# Autodesk Inventor assembly: Nozzle-Brush-Unit
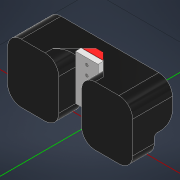
[picture p0: Inventor's stored thumbnail of the model, 180x180]
Saved by Autodesk Inventor 2022.2 (Build 262287010, 287A)
## iProperties
Created: 2022-03-17
Part Number: Nozzle-Brush-Unit
Document SubType Name: Assembly
Designer: sleib
Author: sleib
## Documents named in this file (6)
- C:\Users\sleib\Projekte\Voron-2\CAD\Inventor\Nozzle Brush\Nozzle-Brush-Unit.iam
- C:\Users\sleib\Projekte\Voron-2\CAD\Inventor\Nozzle Brush\Nozzle-Brush Holder (slim).ipt
- C:\Users\sleib\Projekte\Voron-2\CAD\Inventor\Nozzle Brush\Brush Holder Sheet Stop.ipt
- C:\Users\sleib\Projekte\Voron-2\CAD\Inventor\M3x8 SHCS.ipt
- C:\Users\sleib\Projekte\Voron-2\CAD\Inventor\Nozzle Brush\Purge-Bucket.ipt
- C:\Users\sleib\Projekte\Voron-2\CAD\Inventor\Magnet (3x6mm).ipt
## Components (7 placed, 5 different names)
1. Nozzle-Brush Holder (slim):1 — Passend:1, Passend:2, Passend:5, Passend:6, Fluchtend:2
2. Brush Holder Sheet Stop:1 — Passend:1, Passend:2, Passend:3, Passend:4, Passend:7, Passend:8, Passend:14, Fluchtend:1
3. M3x8 SHCS:1 — Passend:3, Passend:5, Passend:8
4. M3x8 SHCS:2 — Passend:4, Passend:6, Passend:7
5. Purge-Bucket:1 — Passend:9, Passend:10, Passend:14, Passend:15, Passend:16, Fluchtend:1, Fluchtend:2
6. Magnet (3x6mm):1 — Passend:9, Passend:16
7. Magnet (3x6mm):2 — Passend:10, Passend:15
## Relationships (15: Mate 13, Flush 2)
- Passend:1 [Mate]: Nozzle-Brush Holder (slim):1 ↔ Brush Holder Sheet Stop:1
- Passend:2 [Mate]: Nozzle-Brush Holder (slim):1 ↔ Brush Holder Sheet Stop:1
- Passend:3 [Mate]: Brush Holder Sheet Stop:1 ↔ M3x8 SHCS:1
- Passend:4 [Mate]: Brush Holder Sheet Stop:1 ↔ M3x8 SHCS:2
- Passend:5 [Mate]: Nozzle-Brush Holder (slim):1 ↔ M3x8 SHCS:1
- Passend:6 [Mate]: Nozzle-Brush Holder (slim):1 ↔ M3x8 SHCS:2
- Passend:7 [Mate]: Brush Holder Sheet Stop:1 ↔ M3x8 SHCS:2
- Passend:8 [Mate]: Brush Holder Sheet Stop:1 ↔ M3x8 SHCS:1
- Passend:9 [Mate]: Purge-Bucket:1 ↔ Magnet (3x6mm):1
- Passend:10 [Mate]: Purge-Bucket:1 ↔ Magnet (3x6mm):2
- Passend:14 [Mate]: Brush Holder Sheet Stop:1 ↔ Purge-Bucket:1
- Passend:15 [Mate]: Purge-Bucket:1 ↔ Magnet (3x6mm):2
- Passend:16 [Mate]: Purge-Bucket:1 ↔ Magnet (3x6mm):1
- Fluchtend:1 [Flush]: Brush Holder Sheet Stop:1 ↔ Purge-Bucket:1
- Fluchtend:2 [Flush]: Nozzle-Brush Holder (slim):1 ↔ Purge-Bucket:1
